# Autodesk Inventor assembly: VP-Input-CIM
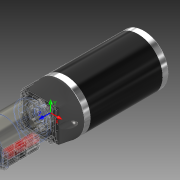
[picture p0: Inventor's stored thumbnail of the model, 180x180]
Saved by Autodesk Inventor 2021 (Build 250183000, 183)
## iProperties
Created: 2018-08-19
Part Number: VP-Input-CIM
Document SubType Name: Assembly
## Documents named in this file (8)
- D:\FIRST\Design\CollabPartsLib\Motors\FRC\Versaplanetary\V2 Stages\CIM Input Stage\VP CIM Input.iam
- D:\FIRST\Design\CollabPartsLib\Motors\FRC\Versaplanetary\Motor Mounting Plates\VP CIM Adapter.ipt
- D:\FIRST\Design\CollabPartsLib\Motors\FRC\Versaplanetary\Input Coupler\Coupler Set Screw.ipt
- D:\FIRST\Design\CollabPartsLib\Motors\FRC\Versaplanetary\Input Coupler\VP Input Coupler.ipt
- D:\FIRST\Design\CollabPartsLib\Motors\FRC\Versaplanetary\Screws\10-32 x .50in Screw.ipt
- D:\FIRST\Design\CollabPartsLib\Motors\FRC\Mini Cim.ipt
- D:\FIRST\Design\CollabPartsLib\Motors\FRC\CIM Motor.ipt
- D:\FIRST\Design\CollabPartsLib\Motors\FRC\Versaplanetary\V2 Stages\CIM Input Stage.iam
## Components (7 placed, 6 different names)
1. VP CIM Adapter:1 — Insert:3, Insert:4
2. CIM Motor:1
3. Coupler Set Screw:1 — Mate:3, Tangent:1
4. VP Input Coupler:1 — Mate:3, Tangent:1
5. 10-32 x .50in Screw:1 — Insert:3
6. 10-32 x .50in Screw:2 — Insert:4
7. Mini Cim:1
## Relationships (8: Insert 4, Mate 3, Tangent 1)
- [Insert]: VP CIM Adapter:1 ↔ CIM Motor:1
- [Insert]: VP CIM Adapter:1 ↔ CIM Motor:1
- [Mate]: CIM Motor:1 ↔ VP Input Coupler:1
- [Mate] (1.1 mm): CIM Motor:1 ↔ VP Input Coupler:1
- Mate:3: Coupler Set Screw:1 ↔ VP Input Coupler:1
- Tangent:1: Coupler Set Screw:1 ↔ VP Input Coupler:1
- Insert:3: VP CIM Adapter:1 ↔ 10-32 x .50in Screw:1
- Insert:4: VP CIM Adapter:1 ↔ 10-32 x .50in Screw:2
